# Autodesk Inventor assembly: Hotend Samling v3
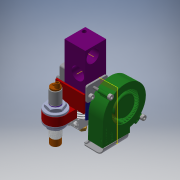
[picture p0: Inventor's stored thumbnail of the model, 180x180]
Saved by Autodesk Inventor 2016 (Build 200138000, 138)
## iProperties
Created: 2015-11-22
Part Number: Hotend Samling v3
Document SubType Name: Assembly
Designer: PowerStation9000
Author: PowerStation9000
## Documents named in this file (16)
- C:\Users\PowerStation9000\AppData\Local\Autodesk\Autodesk Sync\Cloud\mathiaslk\UltiBot mk2 rev2\Egne komponenter\XY Hotend mount\Hotend Samling v3.iam
- C:\Users\PowerStation9000\AppData\Local\Autodesk\Autodesk Sync\Cloud\mathiaslk\UltiBot mk2 rev2\Egne komponenter\XY Hotend mount\Main v3.ipt
- C:\Users\PowerStation9000\AppData\Local\Autodesk\Autodesk Sync\Cloud\mathiaslk\UltiBot mk2 rev2\Importerede komponenter\E3Dv6 Hotend\E3Dv6 Alone.iam
- C:\Users\PowerStation9000\AppData\Local\Autodesk\Autodesk Sync\Cloud\mathiaslk\UltiBot mk2 rev2\Importerede komponenter\E3Dv6 Hotend\v6 Fan Duct.ipt
- C:\Users\PowerStation9000\AppData\Local\Autodesk\Autodesk Sync\Cloud\mathiaslk\UltiBot mk2 rev2\Importerede komponenter\E3Dv6 Hotend\Fan-DC-KDE0503PFB3-Promoco_Fan-DC-KDE0503PFB3-Promoco.iam
- C:\Users\PowerStation9000\AppData\Local\Autodesk\Autodesk Sync\Cloud\mathiaslk\UltiBot mk2 rev2\Egne komponenter\XY Hotend mount\ProbeMount v3.ipt
- C:\Users\PowerStation9000\AppData\Local\Autodesk\Autodesk Sync\Cloud\mathiaslk\UltiBot mk2 rev2\Importerede komponenter\Proxy probe\LJ12A3-4-Z-BY.iam
- C:\Users\PowerStation9000\AppData\Local\Autodesk\Autodesk Sync\Cloud\mathiaslk\UltiBot mk2 rev2\Importerede komponenter\Proxy probe\LJ12A3-4-Z-BY-4.ipt
- C:\Users\PowerStation9000\AppData\Local\Autodesk\Autodesk Sync\Cloud\mathiaslk\UltiBot mk2 rev2\Importerede komponenter\Proxy probe\LJ12A3-4-Z-BY-5.ipt
- C:\Users\PowerStation9000\AppData\Local\Autodesk\Autodesk Sync\Cloud\mathiaslk\UltiBot mk2 rev2\Importerede komponenter\Centrifugal Fan\Fan - USE THIS.ipt
- C:\Users\PowerStation9000\AppData\Local\Autodesk\Autodesk Sync\Cloud\mathiaslk\UltiBot mk2 rev2\Egne komponenter\XY Hotend mount\BlæserMount.ipt
- C:\Users\PowerStation9000\AppData\Local\Autodesk\Autodesk Sync\Cloud\mathiaslk\UltiBot mk2 rev2\Egne komponenter\XY Hotend mount\Hotend Lock 3.ipt
- C:\Users\PowerStation9000\AppData\Local\Autodesk\Autodesk Sync\Cloud\mathiaslk\UltiBot mk2 rev2\Egne komponenter\XY Hotend mount\AS 1420 - 1973 - M3 x 12.ipt
- C:\Users\PowerStation9000\AppData\Local\Autodesk\Autodesk Sync\Cloud\mathiaslk\UltiBot mk2 rev2\Egne komponenter\XY Hotend mount\ANSI B18.3.1M - M3x0,5 x 40(2).ipt
- C:\Users\PowerStation9000\AppData\Local\Autodesk\Autodesk Sync\Cloud\mathiaslk\UltiBot mk2 rev2\Egne komponenter\XY Hotend mount\ANSI B18.3.1M - M3x0,5 x 25(2).ipt
- C:\Users\PowerStation9000\AppData\Local\Autodesk\Autodesk Sync\Cloud\mathiaslk\UltiBot mk2 rev2\Egne komponenter\XY Hotend mount\Luftkanal.ipt
## Components (18 placed, 15 different names)
1. Main v3:1 — Mate:7, Mate:8, Mate:9, Flush:2, Mate:10, Angle:1, Angle:2, Mate:23, Flush:4, Flush:6, Mate:25, Mate:26
2. E3Dv6 Alone:1 [sub-assembly] — Mate:1, Flush:1, Mate:7, Mate:8, Flush:3, Angle:1, Flush:5
3. v6 Fan Duct:1 — Mate:1, Flush:1, Mate:2, Mate:3, Mate:4
4. Fan-DC-KDE0503PFB3-Promoco_Fan-DC-KDE0503PFB3-Promoco:1 [sub-assembly] — Mate:2, Mate:3, Mate:4, Angle:2
5. ProbeMount v3:1 — Mate:9, Flush:2, Mate:10, Mate:16, Mate:18, Mate:19, Angle:3
6. LJ12A3-4-Z-BY:1 [sub-assembly] — Mate:16, Flush:3, Mate:17
7. LJ12A3-4-Z-BY-4:1
8. LJ12A3-4-Z-BY-5:1 — Mate:19
9. LJ12A3-4-Z-BY-4:2 — Mate:17
10. LJ12A3-4-Z-BY-5:2 — Mate:18
11. Fan - USE THIS:1 — Angle:3, Mate:21, Mate:22, Flush:5, Insert:7, Insert:8, Mate:24, Angle:4
12. BlæserMount:1 — Mate:21, Mate:22, Mate:23, Flush:4, Insert:6
13. Hotend Lock 3:1 — Flush:6, Insert:3
14. Luftkanal:1 — Flush:7
15. AS 1420 - Metric M3 x 12:1 — Insert:3
16. Broached Socket Head Cap Screw - Metric M3x0,5 x 40:1 — Insert:6
17. Broached Socket Head Cap Screw - Metric M3x0,5 x 25:1 — Insert:7
18. Broached Socket Head Cap Screw - Metric M3x0,5 x 25:2 — Insert:8
## Relationships (38: Mate 23, Flush 7, Angle 4, Insert 4)
- Mate:1: E3Dv6 Alone:1 ↔ v6 Fan Duct:1
- Flush:1: E3Dv6 Alone:1 ↔ v6 Fan Duct:1
- Mate:2: v6 Fan Duct:1 ↔ Fan-DC-KDE0503PFB3-Promoco_Fan-DC-KDE0503PFB3-Promoco:1
- Mate:3: v6 Fan Duct:1 ↔ Fan-DC-KDE0503PFB3-Promoco_Fan-DC-KDE0503PFB3-Promoco:1
- Mate:4: v6 Fan Duct:1 ↔ Fan-DC-KDE0503PFB3-Promoco_Fan-DC-KDE0503PFB3-Promoco:1
- Mate:7: Main v3:1 ↔ E3Dv6 Alone:1
- Mate:8: Main v3:1 ↔ E3Dv6 Alone:1
- Mate:9: Main v3:1 ↔ ProbeMount v3:1
- Flush:2: Main v3:1 ↔ ProbeMount v3:1
- Mate:10 (-10 mm): Main v3:1 ↔ ProbeMount v3:1
- [Mate]: LJ12A3-4-Z-BY-4:1 ↔ LJ12A3-4-Z-BY-5:1
- [Mate]: LJ12A3-4-Z-BY-4:1 ↔ LJ12A3-4-Z-BY-5:1
- [Mate]: LJ12A3-4-Z-BY:1 ↔ LJ12A3-4-Z-BY-5:1
- [Mate]: LJ12A3-4-Z-BY-4:2 ↔ LJ12A3-4-Z-BY-5:2
- [Mate]: LJ12A3-4-Z-BY-4:2 ↔ LJ12A3-4-Z-BY-5:2
- Mate:16: ProbeMount v3:1 ↔ LJ12A3-4-Z-BY:1
- Flush:3 (1 mm): E3Dv6 Alone:1 ↔ LJ12A3-4-Z-BY:1
- Mate:17: LJ12A3-4-Z-BY:1 ↔ LJ12A3-4-Z-BY-4:2
- Mate:18: ProbeMount v3:1 ↔ LJ12A3-4-Z-BY-5:2
- Mate:19: ProbeMount v3:1 ↔ LJ12A3-4-Z-BY-5:1
- Angle:1 (0 deg): Main v3:1 ↔ E3Dv6 Alone:1
- Angle:2 (90 deg): Main v3:1 ↔ Fan-DC-KDE0503PFB3-Promoco_Fan-DC-KDE0503PFB3-Promoco:1
- Angle:3 (0 deg): ProbeMount v3:1 ↔ Fan - USE THIS:1
- Mate:21: Fan - USE THIS:1 ↔ BlæserMount:1
- Mate:22: Fan - USE THIS:1 ↔ BlæserMount:1
- Mate:23: Main v3:1 ↔ BlæserMount:1
- Flush:4: Main v3:1 ↔ BlæserMount:1
- Flush:5 (-10 mm): E3Dv6 Alone:1 ↔ Fan - USE THIS:1
- Flush:6: Main v3:1 ↔ Hotend Lock 3:1
- Insert:3: Hotend Lock 3:1 ↔ AS 1420 - Metric M3 x 12:1
- Insert:6: BlæserMount:1 ↔ Broached Socket Head Cap Screw - Metric M3x0,5 x 40:1
- Insert:7: Fan - USE THIS:1 ↔ Broached Socket Head Cap Screw - Metric M3x0,5 x 25:1
- Insert:8: Fan - USE THIS:1 ↔ Broached Socket Head Cap Screw - Metric M3x0,5 x 25:2
- Mate:24: Fan - USE THIS:1
- Angle:4 (0 deg): Fan - USE THIS:1
- Flush:7: Luftkanal:1
- Mate:25: Main v3:1
- Mate:26: Main v3:1
## Named parameters: d19_d40 = 0 mm, d20_d41 = 0 mm
